# Autodesk Inventor assembly: complete
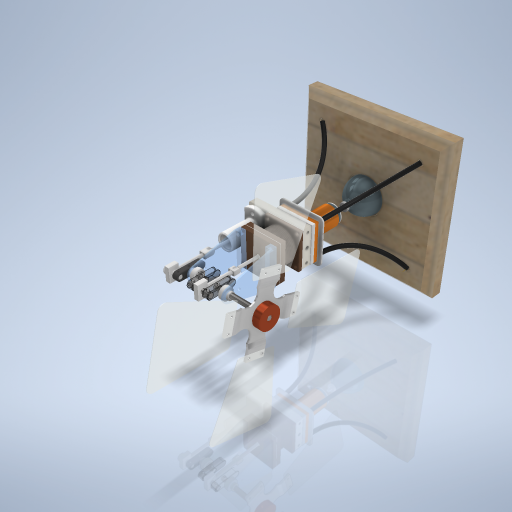
[picture p0: Inventor's stored thumbnail of the model, 512x512]
Saved by Autodesk Inventor 2024.2 (Build 282272000, 272)
## iProperties
Created: 2024-05-16
Part Number: complete
Document SubType Name: Assembly
Designer: Fabri
Author: Fabri
## Documents named in this file (18)
- C:\Users\Fabri\Documents\Inventor\Stirlingfan\complete.iam
- C:\Users\Fabri\Documents\Inventor\Stirlingfan\Support.iam
- C:\Users\Fabri\Documents\Inventor\Stirlingfan\fan.iam
- C:\Users\Fabri\Documents\Inventor\Stirlingfan\BRS_cover.ipt
- C:\Users\Fabri\Documents\Inventor\Stirlingfan\shaft_assembly.iam
- C:\Users\Fabri\Documents\Inventor\Stirlingfan\18.ipt
- C:\Users\Fabri\Documents\Inventor\Stirlingfan\16.ipt
- C:\Users\Fabri\Documents\Inventor\Stirlingfan\17.ipt
- C:\Users\Fabri\Documents\Inventor\Stirlingfan\19.ipt
- C:\Users\Fabri\Documents\Inventor\Stirlingfan\pleuel_small.iam
- C:\Users\Fabri\Documents\Inventor\Stirlingfan\19_1.ipt
- C:\Users\Fabri\Documents\Inventor\Stirlingfan\wing.iam
- C:\Users\Fabri\Documents\Inventor\Stirlingfan\BRS.ipt
- C:\Users\Fabri\Documents\Inventor\Stirlingfan\BMS_support.ipt
- C:\Users\Fabri\Documents\Inventor\Stirlingfan\23.ipt
- C:\Users\Fabri\Documents\Inventor\Stirlingfan\pleuel_big.iam
- C:\Users\Fabri\Documents\Inventor\Stirlingfan\19_2.ipt
- C:\Users\Fabri\Documents\Inventor\Stirlingfan\bolt_shaft.ipt
## Components (18 placed, 17 different names)
1. Support:1 [sub-assembly] — Passend:1, Einfügen:2, Einfügen:10
2. fan:1 [sub-assembly] — Passend:1, Passend:2, Einfügen:3, Einfügen:10, Passend:12, Einfügen:11, Passend:15, Zylindrisch:3
3. BRS_cover:1 — Einfügen:2, Einfügen:9
4. shaft_assembly:1 [sub-assembly] — Passend:2, Einfügen:3, Passend:5, Einfügen:6, Motion, Passend:11, Drehung:1, Einfügen:8, Passend:12, Einfügen:11, Passend:13, Einfügen:12
5. 18:1 — Passend:4, Einfügen:5, Zylindrisch:2
6. 16:1 — Passend:3, Einfügen:4, Passend:4, Einfügen:5
7. 17:1 — Passend:3, Einfügen:4
8. 19:1 — Passend:9, Zylindrisch:2
9. pleuel_small:1 [sub-assembly] — Passend:5, Einfügen:6, Einfügen:7
10. 19_1:1 — Einfügen:7, Passend:10
11. wing:1 [sub-assembly] — Passend:11, Drehung:1, Einfügen:8
12. BRS:1 — Einfügen:9
13. BMS_support:1 — Passend:13, Einfügen:12, Passend:18
14. 23:1 — Passend:15, Zylindrisch:3, Einfügen:14
15. pleuel_big:1 [sub-assembly] — Passend:17, Einfügen:13, Passend:18, Passend:19, Einfügen:15
16. 19_1:2 — Passend:17, Einfügen:13, Drehbar:1
17. 19_2:1 — Drehbar:1, Einfügen:14
18. bolt_shaft:1 — Passend:19, Einfügen:15
## Relationships (33: Mate 14, Insert 14, CylindricalJoint 2, Angle 1, RelateRotation 1, RevoluteJoint 1)
- Passend:1 [Mate]: Support:1 ↔ fan:1
- Einfügen:2 [Insert]: Support:1 ↔ BRS_cover:1
- Passend:2 [Mate]: fan:1 ↔ shaft_assembly:1
- Einfügen:3 [Insert] (-108 mm): fan:1 ↔ shaft_assembly:1
- Passend:3 [Mate]: 16:1 ↔ 17:1
- Einfügen:4 [Insert]: 16:1 ↔ 17:1
- Passend:4 [Mate]: 18:1 ↔ 16:1
- Einfügen:5 [Insert]: 18:1 ↔ 16:1
- Passend:5 [Mate]: shaft_assembly:1 ↔ pleuel_small:1
- Einfügen:6 [Insert] (-17.5 mm): shaft_assembly:1 ↔ pleuel_small:1
- Einfügen:7 [Insert] (-8 mm): pleuel_small:1 ↔ 19_1:1
- Motion [Angle] (450 deg): shaft_assembly:1
- Passend:9 [Mate]: 19:1
- Passend:10 [Mate]: 19_1:1
- Zylindrisch:2 [CylindricalJoint]: 18:1 ↔ 19:1
- Passend:11 [Mate]: shaft_assembly:1 ↔ wing:1
- Drehung:1 [RelateRotation] (1 ul): shaft_assembly:1 ↔ wing:1
- Einfügen:8 [Insert] (-20 mm): shaft_assembly:1 ↔ wing:1
- Einfügen:9 [Insert]: BRS_cover:1 ↔ BRS:1
- Einfügen:10 [Insert] (-10.8 mm): Support:1 ↔ fan:1
- Passend:12 [Mate]: fan:1 ↔ shaft_assembly:1
- Einfügen:11 [Insert] (-108 mm): fan:1 ↔ shaft_assembly:1
- Passend:13 [Mate]: shaft_assembly:1 ↔ BMS_support:1
- Einfügen:12 [Insert] (-8 mm): shaft_assembly:1 ↔ BMS_support:1
- Passend:15 [Mate]: fan:1 ↔ 23:1
- Zylindrisch:3 [CylindricalJoint]: fan:1 ↔ 23:1
- Passend:17 [Mate]: pleuel_big:1 ↔ 19_1:2
- Einfügen:13 [Insert] (-8 mm): pleuel_big:1 ↔ 19_1:2
- Drehbar:1 [RevoluteJoint] (-5.5 mm): 19_1:2 ↔ 19_2:1
- Einfügen:14 [Insert] (-1.5 mm): 23:1 ↔ 19_2:1
- Passend:18 [Mate]: BMS_support:1 ↔ pleuel_big:1
- Passend:19 [Mate]: pleuel_big:1 ↔ bolt_shaft:1
- Einfügen:15 [Insert]: pleuel_big:1 ↔ bolt_shaft:1
